# Autodesk Inventor assembly: Nema 17 Motor a Pasos 17HS4401
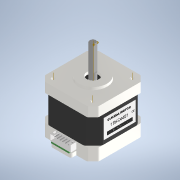
[picture p0: Inventor's stored thumbnail of the model, 180x180]
Saved by Autodesk Inventor 2021 (Build 250183000, 183)
## iProperties
Created: 2020-08-27
Part Number: Nema 17 Motor a Pasos 17HS4401
Document SubType Name: Assembly
Designer: bober
Sending System: Autodesk Translation Framework v9.3.0.1241
Preprocessor: ST-DEVELOPER v18.1
Title: C:/Users/CDMX Electrónica/Google Drive/106.- Jesus Ramirez/Actividades/Diseños 3D curso/Diseño de feder/Nema17/Nema17/Nema 17 Motor a Pasos 17HS4401.step
## Documents named in this file (6)
- D:\Turret\Models\step_motor\Nema 17 Motor a Pasos 17HS4401.iam
- D:\Turret\Models\step_motor\Tornillo v2.ipt
- D:\Turret\Models\step_motor\Pines v2.ipt
- D:\Turret\Models\step_motor\Flecha 17HS4401 v3.ipt
- D:\Turret\Models\step_motor\INF TECNICA 2 v1.ipt
- D:\Turret\Models\step_motor\Part10.ipt
## Components (8 placed, 5 different names)
1. Tornillo v2:1
2. Tornillo v2:2
3. Tornillo v2:3
4. Tornillo v2:4
5. Pines v2:1
6. Flecha 17HS4401 v3:1 — Mate:1, Mate:2
7. INF TECNICA 2 v1:1
8. Part10 — Angle:1, Mate:4, Mate:5, Mate:6, Mate:7
## Relationships (8: Mate 7, Angle 1)
- Mate:1: Flecha 17HS4401 v3:1
- Mate:2: Flecha 17HS4401 v3:1
- Mate:3
- Angle:1 (0 deg): Part10
- Mate:4: Part10
- Mate:5: Part10
- Mate:6: Part10
- Mate:7: Part10
